# Autodesk Inventor assembly: Ensamble de Piezas
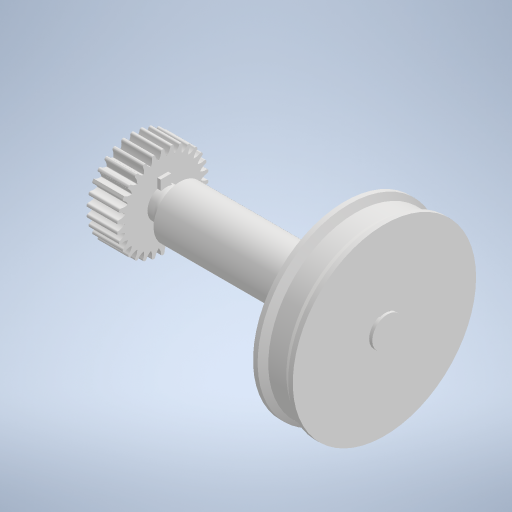
[picture p0: Inventor's stored thumbnail of the model, 512x512]
Saved by Autodesk Inventor 2024.2 (Build 282272000, 272)
## iProperties
Created: 2024-03-31
Part Number: Ensamble de Piezas
Document SubType Name: Assembly
Designer: Josh Juárez
Author: Josh Juárez
## Documents named in this file (5)
- D:\Universidad\Ciclo #5\Dinámica LAB\Tarea Ensamble\Ensamble de Piezas.iam
- C:\Users\Josh Juárez\Downloads\CUÑA.ipt
- C:\Users\Josh Juárez\Downloads\POLEA.ipt
- C:\Users\Josh Juárez\Downloads\ENGRANE.ipt
- C:\Users\Josh Juárez\Downloads\EJE_CUÑEROS.ipt
## Components (5 placed, 4 different names)
1. POLEA:1 — Mate:2, Flush:1
2. ENGRANE:1 — Mate:1
3. EJE_CUÑEROS:1 — Rigid:1, Rigid:2, Mate:1, Mate:2
4. CUÑA:3 — Rigid:1, Flush:1
5. CUÑA:4 — Rigid:2
## Relationships (5: WeldJoint 2, Mate 2, Flush 1)
- Rigid:1 [WeldJoint]: EJE_CUÑEROS:1 ↔ CUÑA:3
- Rigid:2 [WeldJoint]: EJE_CUÑEROS:1 ↔ CUÑA:4
- Mate:1: ENGRANE:1 ↔ EJE_CUÑEROS:1
- Mate:2: POLEA:1 ↔ EJE_CUÑEROS:1
- Flush:1: POLEA:1 ↔ CUÑA:3
